# Autodesk Inventor assembly: FE-00007
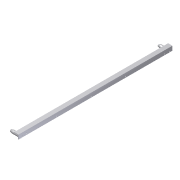
[picture p0: Inventor's stored thumbnail of the model, 180x180]
Saved by Autodesk Inventor 2012 (Build 160160000, 160)
## iProperties
Created: 2008-05-27
Part Number: FE-00007
Description: Field Top Rail Assy
Document SubType Name: Assembly
Designer: narosenberg
Author: narosenberg
## Documents named in this file (4)
- C:\Data Folder\FRC 2012 Field\Components\FE-00007.iam
- C:\Data Folder\FRC 2012 Field\Components\FE-00007-01.ipt
- C:\Data Folder\FRC 2012 Field\Components\FE-00007-02.ipt
- C:\Data Folder\FRC 2012 Field\Components\FE-00007-03.ipt
## Components (4 placed, 3 different names)
1. FE-00007-01:1 — Mate:1, Flush:1, Flush:2
2. FE-00007-02:1 — Mate:1, Flush:1, Flush:2
3. FE-00007-03:1
4. FE-00007-03:2
## Relationships (5: Flush 2, Insert 2, Mate 1)
- Mate:1: FE-00007-01:1 ↔ FE-00007-02:1
- Flush:1: FE-00007-01:1 ↔ FE-00007-02:1
- Flush:2 (-75.4062 mm): FE-00007-01:1 ↔ FE-00007-02:1
- [Insert]: FE-00007-01:1 ↔ FE-00007-03:2
- [Insert]: FE-00007-01:1 ↔ FE-00007-03:1
